# Autodesk Inventor assembly: Left Hook Encoder Assembly
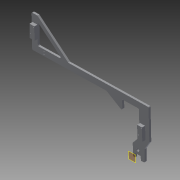
[picture p0: Inventor's stored thumbnail of the model, 180x180]
Saved by Autodesk Inventor 2013 (Build 170138000, 138)
## iProperties
Created: 2013-03-16
Part Number: Left Hook Encoder Assembly
Document SubType Name: Assembly
Designer: Arpan
Author: Arpan
## Documents named in this file (3)
- C:\Users\Arpan\Documents\GitHub\frc2013CAD\Midwest Climber\Left Hook Encoder Assembly.iam
- C:\Users\Arpan\Documents\GitHub\frc2013CAD\Midwest Climber\Limit Switch.ipt
- C:\Users\Arpan\Documents\GitHub\frc2013CAD\Midwest Climber\Left Climber Hook_v2.ipt
## Components (3 placed, 2 different names)
1. Limit Switch:1 — Mate:3, Angle:1, Mate:5
2. Left Climber Hook_v2:1 — Mate:3, Angle:1, Mate:4, Mate:5, Mate:6, Angle:2
3. Limit Switch:2 — Mate:4, Mate:6, Angle:2
## Relationships (6: Mate 4, Angle 2)
- Mate:3: Limit Switch:1 ↔ Left Climber Hook_v2:1
- Angle:1 (0 deg): Limit Switch:1 ↔ Left Climber Hook_v2:1
- Mate:4: Left Climber Hook_v2:1 ↔ Limit Switch:2
- Mate:5: Limit Switch:1 ↔ Left Climber Hook_v2:1
- Mate:6: Left Climber Hook_v2:1 ↔ Limit Switch:2
- Angle:2 (0 deg): Left Climber Hook_v2:1 ↔ Limit Switch:2
